# Autodesk Inventor assembly: Electromanetic brake
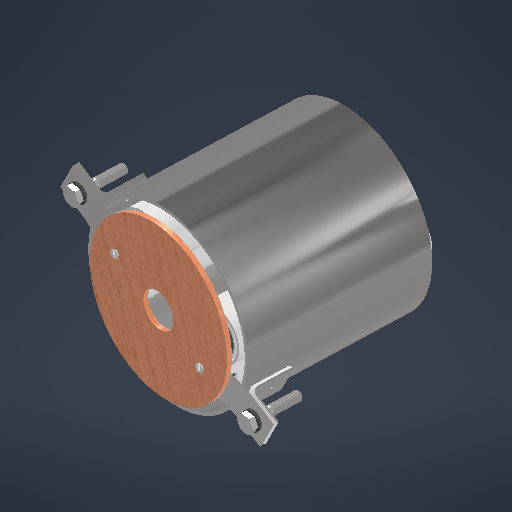
[picture p0: Inventor's stored thumbnail of the model, 512x512]
Saved by Autodesk Inventor 2026.3 (Build 303398000, 398)
## iProperties
Created: 2026-08-09
Part Number: Electromanetic brake
Document SubType Name: Assembly
Designer: matot
Author: matot
## Documents named in this file (8)
- C:\Users\matot\OneDrive - Stellenbosch University\2026\MechatronicsProject478\Building the joint\Joint Assembly\Electromanetic brake.iam
- C:\Users\matot\OneDrive - Stellenbosch University\2026\MechatronicsProject478\Building the joint\Joint Assembly\Electromagnet final_key.iam
- C:\Users\matot\OneDrive - Stellenbosch University\2026\MechatronicsProject478\Building the joint\Joint Assembly\Pressure platform.ipt
- C:\Users\matot\OneDrive - Stellenbosch University\2026\MechatronicsProject478\Building the joint\Joint Assembly\Friction Plate.ipt
- C:\Users\matot\OneDrive - Stellenbosch University\Documents\Inventor\Content Center Files\R2026\en-US\ISO 4036(2)\ISO 4036 - M4(2).ipt
- C:\Users\matot\OneDrive - Stellenbosch University\Documents\Inventor\Content Center Files\R2026\en-US\ISO 2009(2)\ISO 2009 - M3 x 5 - 2.35 - ISO.ipt
- C:\Users\matot\OneDrive - Stellenbosch University\Documents\Inventor\Content Center Files\R2026\en-US\ISO 7091\ISO 7091 - ST 6 - 100 HV.ipt
- C:\Users\matot\OneDrive - Stellenbosch University\Documents\Inventor\Content Center Files\R2026\en-US\ISO 4014(2)\ISO 4014 - M6 x 30 - ISO.ipt
## Components (12 placed, 7 different names)
1. Electromagnet final_key:1 [sub-assembly] — Insert:5, Flush:1, Flush:2, Insert:6, Flush:3
2. Friction Plate:1 — Insert:3, Insert:4, Mate:1, Mate:2, Mate:3, Mate:4
3. Pressure platform:1 — Insert:2, Insert:3, Insert:6, Flush:3, Mate:3, Insert:7
4. Pressure platform:2 — Insert:1, Insert:4, Insert:5, Flush:1, Flush:2, Mate:4, Insert:8
5. ISO 4036 M4:1 — Insert:1
6. ISO 4036 M4:2 — Insert:2
7. ISO 2009 M3 x 5 x 2.35:1 — Mate:1
8. ISO 2009 M3 x 5 x 2.35:2 — Mate:2
9. ISO 7091 ST 6 - 100 HV:1 — Insert:7, Insert:9
10. ISO 7091 ST 6 - 100 HV:2 — Insert:8, Insert:10
11. ISO 4014 M6 x 30:1 — Insert:9
12. ISO 4014 M6 x 30:2 — Insert:10
## Relationships (17: Insert 10, Mate 4, Flush 3)
- Insert:1: Pressure platform:2 ↔ ISO 4036 M4:1
- Insert:2: Pressure platform:1 ↔ ISO 4036 M4:2
- Insert:3: Friction Plate:1 ↔ Pressure platform:1
- Insert:4: Friction Plate:1 ↔ Pressure platform:2
- Mate:1: Friction Plate:1 ↔ ISO 2009 M3 x 5 x 2.35:1
- Mate:2: Friction Plate:1 ↔ ISO 2009 M3 x 5 x 2.35:2
- Insert:5: Electromagnet final_key:1 ↔ Pressure platform:2
- Flush:1: Electromagnet final_key:1 ↔ Pressure platform:2
- Flush:2: Electromagnet final_key:1 ↔ Pressure platform:2
- Insert:6: Electromagnet final_key:1 ↔ Pressure platform:1
- Flush:3: Electromagnet final_key:1 ↔ Pressure platform:1
- Mate:3: Friction Plate:1 ↔ Pressure platform:1
- Mate:4: Friction Plate:1 ↔ Pressure platform:2
- Insert:7: Pressure platform:1 ↔ ISO 7091 ST 6 - 100 HV:1
- Insert:8: Pressure platform:2 ↔ ISO 7091 ST 6 - 100 HV:2
- Insert:9: ISO 7091 ST 6 - 100 HV:1 ↔ ISO 4014 M6 x 30:1
- Insert:10: ISO 7091 ST 6 - 100 HV:2 ↔ ISO 4014 M6 x 30:2
